# Autodesk Inventor assembly: 4C8135
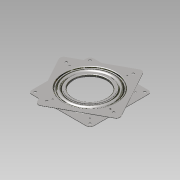
[picture p0: Inventor's stored thumbnail of the model, 180x180]
Saved by Autodesk Inventor 2020.1 (Build 241239000, 239)
## iProperties
Created: 2019-12-09
Document SubType Name: Assembly
Designer: Autodesk Inc.
Catalog Web Link: https://www.triangleoshkosh.com/lazy-susan-turntable-bearing-4c
Vendor: Triangle Mfg.
Company: Autodesk Inc.
Category: FIRSTChoice
Author: Autodesk Inc.
## Documents named in this file (4)
- D:\FIRST 2020\FRC 2020\FRC FIRSTChoice 2020\Inventor\4C8135.iam
- D:\FIRST 2020\FRC 2020\FRC FIRSTChoice 2020\Inventor\Parts\MSTR 4 Inch Locking Race_7719a.ipt
- D:\FIRST 2020\FRC 2020\FRC FIRSTChoice 2020\Inventor\Parts\MSTR 4 Inch Plain Race_2823.ipt
- D:\FIRST 2020\FRC 2020\FRC FIRSTChoice 2020\Inventor\Parts\MSTR Suzie Ball_Balls4.ipt
## Components (38 placed, 38 different names)
1. MSTR 4 Inch Locking Race_7719a_1 — Insert:1
2. MSTR 4 Inch Plain Race_2823_2 — Insert:1
3. MSTR Suzie Ball_Balls4_3
4. MSTR Suzie Ball_Balls4_4
5. MSTR Suzie Ball_Balls4_5
6. MSTR Suzie Ball_Balls4_6
7. MSTR Suzie Ball_Balls4_7
8. MSTR Suzie Ball_Balls4_8
9. MSTR Suzie Ball_Balls4_9
10. MSTR Suzie Ball_Balls4_10
11. MSTR Suzie Ball_Balls4_11
12. MSTR Suzie Ball_Balls4_12
13. MSTR Suzie Ball_Balls4_13
14. MSTR Suzie Ball_Balls4_14
15. MSTR Suzie Ball_Balls4_15
16. MSTR Suzie Ball_Balls4_16
17. MSTR Suzie Ball_Balls4_17
18. MSTR Suzie Ball_Balls4_18
19. MSTR Suzie Ball_Balls4_19
20. MSTR Suzie Ball_Balls4_20
21. MSTR Suzie Ball_Balls4_21
22. MSTR Suzie Ball_Balls4_22
23. MSTR Suzie Ball_Balls4_23
24. MSTR Suzie Ball_Balls4_24
25. MSTR Suzie Ball_Balls4_25
26. MSTR Suzie Ball_Balls4_26
27. MSTR Suzie Ball_Balls4_27
28. MSTR Suzie Ball_Balls4_28
29. MSTR Suzie Ball_Balls4_29
30. MSTR Suzie Ball_Balls4_30
31. MSTR Suzie Ball_Balls4_31
32. MSTR Suzie Ball_Balls4_32
33. MSTR Suzie Ball_Balls4_33
34. MSTR Suzie Ball_Balls4_34
35. MSTR Suzie Ball_Balls4_35
36. MSTR Suzie Ball_Balls4_36
37. MSTR Suzie Ball_Balls4_37
38. MSTR Suzie Ball_Balls4_38
## Relationships (1: Insert 1)
- Insert:1 (-7.3914 mm): MSTR 4 Inch Locking Race_7719a_1 ↔ MSTR 4 Inch Plain Race_2823_2
